# Autodesk Inventor assembly: Hilfsbaugruppe Kantensensor für Zeichnung
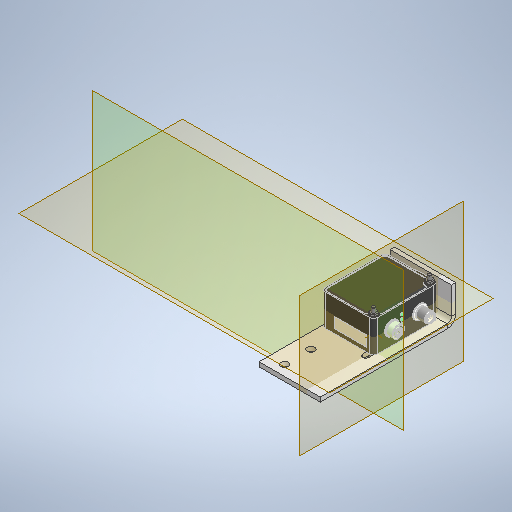
[picture p0: Inventor's stored thumbnail of the model, 512x512]
Saved by Autodesk Inventor 2025.2 (Build 292293000, 293)
## iProperties
Created: 2025-06-24
Part Number: Hilfsbaugruppe Kantensensor für Zeichnung
Document SubType Name: Assembly
Designer: Jakob
Author: Jakob
## Documents named in this file (7)
- D:\Useless_Box\CAD-Paspa\Useless Box\Zeichnung_JH\Hilfsbaugruppe Kantensensor für Zeichnung.iam
- D:\Useless_Box\CAD-Paspa\Useless Box\Kaufteile\BAUMER_BaumerOXS200117288451\AIS2024\Baumer_OXS200_11728845_1.iam
- D:\Useless_Box\CAD-Paspa\Useless Box\Eigene Bauteile\ER_Halterung_Kantensensor.ipt
- D:\Useless_Box\CAD-Paspa\Useless Box\Standart Bauteile\DIN EN ISO 4026 - M5 x 25.ipt
- D:\Useless_Box\CAD-Paspa\Useless Box\Standart Bauteile\DIN 6912 - M4 x 50.ipt
- D:\Useless_Box\CAD-Paspa\Useless Box\Standart Bauteile\DIN EN ISO 4036 - M4.ipt
- D:\Useless_Box\CAD-Paspa\Useless Box\Standart Bauteile\DIN 125 - A 4,3.ipt
## Components (12 placed, 6 different names)
1. Baumer_OXS200_11728845_1:1 [sub-assembly] — Passend:1, Passend:2, Fluchtend:1, Passend:3, Fluchtend:2, Fluchtend:3, Passend:6, Passend:7, Passend:8, Passend:10, Passend:11, Passend:12, Passend:18, Passend:19
2. ER_Halterung_Kantensensor:1 — Passend:3, Fluchtend:2, Fluchtend:3, Passend:4, Passend:5, Passend:9, Passend:14
3. DIN EN ISO 4026 - M5 x 25:1 — Passend:4, Passend:6, Winkel:1
4. DIN EN ISO 4026 - M5 x 25:2 — Passend:5, Passend:7, Winkel:2
5. DIN 6912 - M4 x 50:1 — Passend:11, Passend:13, Passend:16, Passend:20
6. DIN 6912 - M4 x 50:2 — Passend:12, Passend:15, Passend:17, Passend:21
7. DIN EN ISO 4036 - M4:1 — Passend:20, Passend:22
8. DIN EN ISO 4036 - M4:2 — Passend:21, Passend:23
9. DIN 125 - A 4,3:1 — Passend:16, Passend:18, Passend:22
10. DIN 125 - A 4,3:2 — Passend:17, Passend:19, Passend:23
11. DIN 125 - A 4,3:3 — Passend:8, Passend:9, Passend:13
12. DIN 125 - A 4,3:4 — Passend:10, Passend:14, Passend:15
## Relationships (28: Mate 23, Flush 3, Angle 2)
- Passend:1 [Mate]: Baumer_OXS200_11728845_1:1
- Passend:2 [Mate]: Baumer_OXS200_11728845_1:1
- Fluchtend:1 [Flush]: Baumer_OXS200_11728845_1:1
- Passend:3 [Mate] (5 mm): Baumer_OXS200_11728845_1:1 ↔ ER_Halterung_Kantensensor:1
- Fluchtend:2 [Flush]: Baumer_OXS200_11728845_1:1 ↔ ER_Halterung_Kantensensor:1
- Fluchtend:3 [Flush]: Baumer_OXS200_11728845_1:1 ↔ ER_Halterung_Kantensensor:1
- Passend:4 [Mate]: ER_Halterung_Kantensensor:1 ↔ DIN EN ISO 4026 - M5 x 25:1
- Passend:5 [Mate]: ER_Halterung_Kantensensor:1 ↔ DIN EN ISO 4026 - M5 x 25:2
- Passend:6 [Mate]: Baumer_OXS200_11728845_1:1 ↔ DIN EN ISO 4026 - M5 x 25:1
- Passend:7 [Mate]: Baumer_OXS200_11728845_1:1 ↔ DIN EN ISO 4026 - M5 x 25:2
- Passend:8 [Mate]: Baumer_OXS200_11728845_1:1 ↔ DIN 125 - A 4,3:3
- Passend:9 [Mate]: ER_Halterung_Kantensensor:1 ↔ DIN 125 - A 4,3:3
- Passend:10 [Mate]: Baumer_OXS200_11728845_1:1 ↔ DIN 125 - A 4,3:4
- Passend:11 [Mate]: Baumer_OXS200_11728845_1:1 ↔ DIN 6912 - M4 x 50:1
- Passend:12 [Mate]: Baumer_OXS200_11728845_1:1 ↔ DIN 6912 - M4 x 50:2
- Passend:13 [Mate]: DIN 6912 - M4 x 50:1 ↔ DIN 125 - A 4,3:3
- Passend:14 [Mate]: ER_Halterung_Kantensensor:1 ↔ DIN 125 - A 4,3:4
- Passend:15 [Mate]: DIN 6912 - M4 x 50:2 ↔ DIN 125 - A 4,3:4
- Passend:16 [Mate]: DIN 6912 - M4 x 50:1 ↔ DIN 125 - A 4,3:1
- Passend:17 [Mate]: DIN 6912 - M4 x 50:2 ↔ DIN 125 - A 4,3:2
- Passend:18 [Mate]: Baumer_OXS200_11728845_1:1 ↔ DIN 125 - A 4,3:1
- Passend:19 [Mate]: Baumer_OXS200_11728845_1:1 ↔ DIN 125 - A 4,3:2
- Passend:20 [Mate]: DIN 6912 - M4 x 50:1 ↔ DIN EN ISO 4036 - M4:1
- Passend:21 [Mate]: DIN 6912 - M4 x 50:2 ↔ DIN EN ISO 4036 - M4:2
- Passend:22 [Mate]: DIN EN ISO 4036 - M4:1 ↔ DIN 125 - A 4,3:1
- Passend:23 [Mate]: DIN EN ISO 4036 - M4:2 ↔ DIN 125 - A 4,3:2
- Winkel:1 [Angle] (0 deg): DIN EN ISO 4026 - M5 x 25:1
- Winkel:2 [Angle] (0 deg): DIN EN ISO 4026 - M5 x 25:2
